# Autodesk Inventor assembly: 5mm_cnc_v1
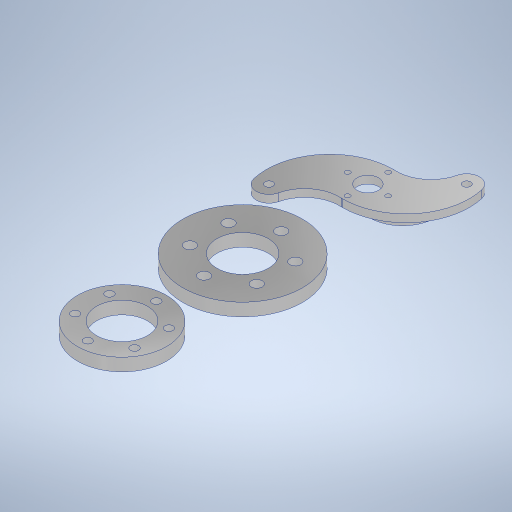
[picture p0: Inventor's stored thumbnail of the model, 512x512]
Saved by Autodesk Inventor 2024.3 (Build 283343010, 343A)
## iProperties
Created: 2025-07-03
Part Number: 5mm_cnc_v1
Document SubType Name: Assembly
Designer: kshau
Author: kshau
## Documents named in this file (4)
- C:\Users\kshau\Documents\inventor\Create_ViperX\FlatPattern\5mm_cnc_v1.iam
- C:\Users\kshau\Documents\inventor\Create_ViperX\UpperArm_Component\servohorn_forR0.ipt
- C:\Users\kshau\Documents\inventor\Create_ViperX\Base_Component\servoplate_forR3.ipt
- C:\Users\kshau\Documents\inventor\Create_ViperX\ViperX_hand\rotor.ipt
## Components (3 placed, 3 different names)
1. servohorn_forR0:1
2. servoplate_forR3:1 — フラッシュ:1
3. rotor:1 — フラッシュ:1
## Relationships (1: Flush 1)
- フラッシュ:1 [Flush]: servoplate_forR3:1 ↔ rotor:1
